# Autodesk Inventor assembly: crane assembly
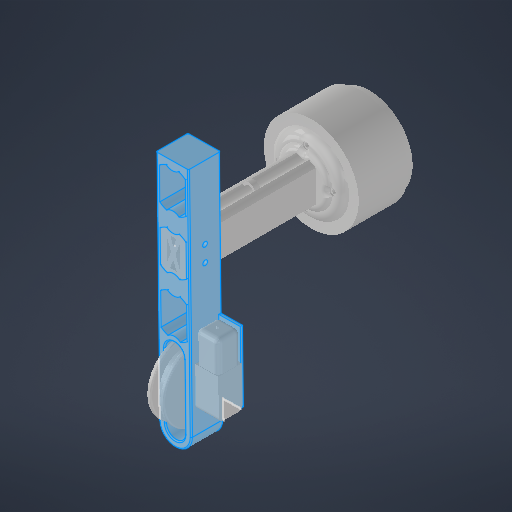
[picture p0: Inventor's stored thumbnail of the model, 512x512]
Saved by Autodesk Inventor 2026.2 (Build 302298010, 298A)
## iProperties
Created: 2026-02-27
Part Number: crane assembly
Document SubType Name: Assembly
Designer: AdminForWorker
Title: crane assembly v5
Author: AdminForWorker
## Documents named in this file (7)
- C:\Users\bobmi\OneDrive - Heriot-Watt University\Github\System-Project-G2\mechanical\crane-assembly-group2.iam
- C:\Users\bobmi\OneDrive - Heriot-Watt University\Github\System-Project-G2\mechanical\crane\horizontal-crane-component-group2.ipt
- C:\Users\bobmi\OneDrive - Heriot-Watt University\Github\System-Project-G2\mechanical\crane\spool-group2.ipt
- C:\Users\bobmi\OneDrive - Heriot-Watt University\Github\System-Project-G2\mechanical\buggy\motor-group2.ipt
- C:\Users\bobmi\OneDrive - Heriot-Watt University\Github\System-Project-G2\mechanical\crane\vertical-crane-component-group2.ipt
- C:\Users\bobmi\OneDrive - Heriot-Watt University\Github\System-Project-G2\mechanical\crane\rotating-base-bottom-group2.ipt
- C:\Users\bobmi\OneDrive - Heriot-Watt University\Github\System-Project-G2\mechanical\crane\rotating-base-head-group2.ipt
## Components (6 placed, 6 different names)
1. Horizontal arm component v4:1 — Rigid:1, Mate:1, Flush:1, Mate:2
2. spool v3:1 — Insert:1
3. MOTOR v3:1 — Mate:1, Flush:1, Mate:2, Insert:1
4. crane vertical component_ v3:1 — Rigid:1, Mate:4, Mate:5
5. rotating-base-bottom-group2:1 — Flush:2, Flush:3, Mate:3, Insert:2
6. rotating-base-head-group2:1 — Insert:2, Crane rotation, Mate:4
## Relationships (12: Mate 5, Flush 3, Insert 2, WeldJoint 1, Angle 1)
- Rigid:1 [WeldJoint]: Horizontal arm component v4:1 ↔ crane vertical component_ v3:1
- Mate:1: Horizontal arm component v4:1 ↔ MOTOR v3:1
- Flush:1: Horizontal arm component v4:1 ↔ MOTOR v3:1
- Mate:2: Horizontal arm component v4:1 ↔ MOTOR v3:1
- Insert:1 (-3 mm): spool v3:1 ↔ MOTOR v3:1
- Flush:2: rotating-base-bottom-group2:1
- Flush:3: rotating-base-bottom-group2:1
- Mate:3: rotating-base-bottom-group2:1
- Insert:2: rotating-base-bottom-group2:1 ↔ rotating-base-head-group2:1
- Crane rotation [Angle] (0 deg): rotating-base-head-group2:1
- Mate:4: crane vertical component_ v3:1 ↔ rotating-base-head-group2:1
- Mate:5: crane vertical component_ v3:1
